# Autodesk Inventor assembly: Head
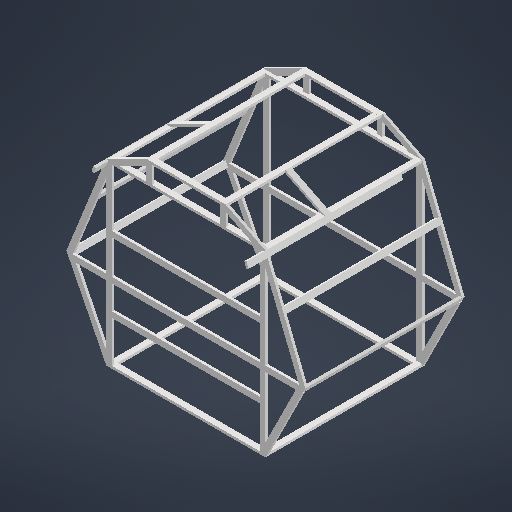
[picture p0: Inventor's stored thumbnail of the model, 512x512]
Saved by Autodesk Inventor 2026 (Build 300175000, 175)
## iProperties
Created: 2025-09-02
Part Number: Head
Document SubType Name: Assembly
Designer: trott
Author: trott
## Documents named in this file (12)
- C:\Users\trott\Documents\UofSC-ASME-Tiger-Burn-Design-2025\CAD\Head\Head.iam
- C:\Users\trott\Documents\UofSC-ASME-Tiger-Burn-Design-2025\CAD\Head\2x4x96.ipt
- C:\Users\trott\Documents\UofSC-ASME-Tiger-Burn-Design-2025\CAD\Head\2x4x89.ipt
- C:\Users\trott\Documents\UofSC-ASME-Tiger-Burn-Design-2025\CAD\Head\2x4x105.ipt
- C:\Users\trott\Documents\UofSC-ASME-Tiger-Burn-Design-2025\CAD\Head\S_2x4x24.ipt
- C:\Users\trott\Documents\UofSC-ASME-Tiger-Burn-Design-2025\CAD\Head\S_2x4x64.622.ipt
- C:\Users\trott\Documents\UofSC-ASME-Tiger-Burn-Design-2025\CAD\Head\S_2x4x48.13.ipt
- C:\Users\trott\Documents\UofSC-ASME-Tiger-Burn-Design-2025\CAD\Head\2x4x48.ipt
- C:\Users\trott\Documents\UofSC-ASME-Tiger-Burn-Design-2025\CAD\Head\2x4x10.5.ipt
- C:\Users\trott\Documents\UofSC-ASME-Tiger-Burn-Design-2025\CAD\Head\S_2x4x26.833.ipt
- C:\Users\trott\Documents\UofSC-ASME-Tiger-Burn-Design-2025\CAD\Head\2x4x93.ipt
- C:\Users\trott\Documents\UofSC-ASME-Tiger-Burn-Design-2025\CAD\Head\S2_2x4x26.833.ipt
## Components (48 placed, 11 different names)
1. 2x4x89:5 — Mate:5, Flush:11, Flush:12, Flush:14, Flush:15, Flush:18, Flush:23, Flush:24, Flush:49, Flush:52
2. 2x4x89:6 — Mate:6, Flush:13, Flush:14
3. S_2x4x64.622:1 — Mate:9, Flush:19
4. S_2x4x64.622:2 — Mate:10, Flush:20, Mate:46, Flush:58
5. S_2x4x64.622:3 — Mate:11, Mate:12, Flush:21, Mate:41, Mate:45, Flush:57
6. S_2x4x64.622:4 — Mate:13, Mate:14
7. S_2x4x48.13:1 — Mate:15, Flush:22, Mate:16
8. S_2x4x48.13:2 — Mate:17, Flush:25
9. S_2x4x48.13:3 — Mate:18, Mate:19, Flush:26, Mate:40
10. S_2x4x48.13:4 — Mate:20, Mate:21, Flush:27
11. 2x4x10.5:1 — Mate:22, Flush:28, Flush:32, Flush:39, Flush:40, Mate:27, Flush:46
12. 2x4x10.5:2 — Mate:23, Flush:29, Flush:31, Flush:45
13. 2x4x10.5:3 — Mate:24, Flush:34, Flush:35, Flush:38, Flush:47
14. 2x4x10.5:4 — Mate:25, Flush:33, Flush:36, Flush:37, Mate:26, Flush:48
15. 2x4x48:1 — Flush:37, Flush:38, Mate:26, Flush:41, Mate:28, Flush:42, Mate:33, Mate:35
16. 2x4x48:2 — Flush:39, Flush:40, Mate:27, Flush:43, Flush:44, Mate:29, Mate:30, Mate:31
17. 2x4x89:7 — Flush:41, Mate:28, Flush:42, Mate:43
18. 2x4x89:8 — Flush:43, Flush:44, Mate:29, Mate:42
19. S_2x4x26.833:1 — Flush:45, Mate:30, Flush:56
20. S_2x4x26.833:2 — Mate:31, Mate:32, Flush:46, Flush:55
21. S_2x4x26.833:3 — Mate:33, Mate:34, Flush:47
22. S_2x4x26.833:4 — Mate:35, Flush:48
23. 2x4x89:9 — Mate:36, Flush:49, Flush:50
24. 2x4x89:10 — Mate:37, Flush:51, Flush:52
25. 2x4x93:1 — Mate:38, Mate:39, Flush:53
26. 2x4x93:2 — Mate:40, Mate:41, Flush:54
27. S2_2x4x26.833:1 — Mate:42, Flush:56
28. S2_2x4x26.833:2 — Mate:43, Mate:44, Flush:55
29. 2x4x93:3 — Mate:45, Flush:57, Flush:64
30. 2x4x93:4 — Mate:46, Flush:58, Flush:63
31. 2x4x93:5 — Mate:51, Flush:63
32. 2x4x93:6 — Mate:52, Flush:64
33. 2x4x105:1 — Mate:4, Flush:9, Flush:10, Mate:5, Flush:11, Mate:8, Flush:17, Mate:19, Flush:26, Mate:36
34. 2x4x105:2 — Mate:6, Flush:13, Mate:20, Flush:27
35. 2x4x105:3 — Mate:7, Flush:16, Flush:22, Flush:50, Mate:37, Flush:51
36. 2x4x105:4 — Flush:25
37. 2x4x96:1 — Mate:1, Flush:1, Flush:2, Mate:2, Flush:3, Flush:4, Mate:4, Flush:9, Flush:10, Mate:21
38. 2x4x89:1 — Mate:1, Flush:1, Flush:2, Flush:8
39. 2x4x89:2 — Mate:2, Flush:3, Flush:4, Flush:5, Mate:3, Flush:6, Flush:7, Flush:12
40. 2x4x96:2 — Flush:5, Mate:3, Flush:6, Flush:7, Flush:8, Mate:15, Mate:16
41. 2x4x96:3 — Mate:12, Mate:13, Flush:32, Flush:35, Mate:32, Mate:34, Mate:44, Mate:52
42. 2x4x89:3 — Mate:24, Mate:25, Flush:33, Flush:34
43. 2x4x89:4 — Mate:22, Mate:23, Flush:28, Flush:29
44. 2x4x96:4 — Flush:31, Flush:36, Mate:51
45. S_2x4x24:2 — Mate:8, Flush:17, Flush:18, Mate:11, Flush:21, Flush:24, Mate:18, Flush:54
46. S_2x4x24:1 — Mate:7, Flush:15, Flush:16, Mate:10, Flush:20, Flush:23, Mate:38, Mate:39, Flush:53
47. S_2x4x24:3 — Mate:14
48. S_2x4x24:4 — Mate:9, Flush:19, Mate:17
## Component patterns: (4 elements, first: 2x4x105:1), (2 elements, first: 2x4x96:1 + 2x4x89:1 + 2x4x89:2 + 2x4x96:2), (2 elements, first: S_2x4x24:2 + S_2x4x24:1)
## Relationships (107: Flush 59, Mate 48)
- Mate:1: 2x4x96:1 ↔ 2x4x89:1
- Flush:1: 2x4x96:1 ↔ 2x4x89:1
- Flush:2: 2x4x96:1 ↔ 2x4x89:1
- Mate:2: 2x4x96:1 ↔ 2x4x89:2
- Flush:3: 2x4x96:1 ↔ 2x4x89:2
- Flush:4: 2x4x96:1 ↔ 2x4x89:2
- Flush:5: 2x4x89:2 ↔ 2x4x96:2
- Mate:3: 2x4x89:2 ↔ 2x4x96:2
- Flush:6: 2x4x89:2 ↔ 2x4x96:2
- Flush:7: 2x4x89:2 ↔ 2x4x96:2
- Flush:8: 2x4x89:1 ↔ 2x4x96:2
- Mate:4: 2x4x105:1 ↔ 2x4x96:1
- Flush:9: 2x4x105:1 ↔ 2x4x96:1
- Flush:10: 2x4x105:1 ↔ 2x4x96:1
- Mate:5: 2x4x89:5 ↔ 2x4x105:1
- Flush:11: 2x4x89:5 ↔ 2x4x105:1
- Flush:12 (1130.3 mm): 2x4x89:5 ↔ 2x4x89:2
- Mate:6: 2x4x89:6 ↔ 2x4x105:2
- Flush:13: 2x4x89:6 ↔ 2x4x105:2
- Flush:14: 2x4x89:5 ↔ 2x4x89:6
- Mate:7: 2x4x105:3 ↔ S_2x4x24:1
- Flush:15: 2x4x89:5 ↔ S_2x4x24:1
- Flush:16: 2x4x105:3 ↔ S_2x4x24:1
- Mate:8: 2x4x105:1 ↔ S_2x4x24:2
- Flush:17: 2x4x105:1 ↔ S_2x4x24:2
- Flush:18: 2x4x89:5 ↔ S_2x4x24:2
- Mate:9: S_2x4x64.622:1 ↔ S_2x4x24:4
- Flush:19: S_2x4x64.622:1 ↔ S_2x4x24:4
- Mate:10: S_2x4x64.622:2 ↔ S_2x4x24:1
- Flush:20: S_2x4x64.622:2 ↔ S_2x4x24:1
- Mate:11: S_2x4x64.622:3 ↔ S_2x4x24:2
- Mate:12: S_2x4x64.622:3 ↔ 2x4x96:3
- Flush:21: S_2x4x64.622:3 ↔ S_2x4x24:2
- Mate:13: S_2x4x64.622:4 ↔ 2x4x96:3
- Mate:14: S_2x4x64.622:4 ↔ S_2x4x24:3
- Mate:15: S_2x4x48.13:1 ↔ 2x4x96:2
- Flush:22: S_2x4x48.13:1 ↔ 2x4x105:3
- Mate:16: S_2x4x48.13:1 ↔ 2x4x96:2
- Flush:23: 2x4x89:5 ↔ S_2x4x24:1
- Flush:24: 2x4x89:5 ↔ S_2x4x24:2
- Mate:17: S_2x4x48.13:2 ↔ S_2x4x24:4
- Flush:25: S_2x4x48.13:2 ↔ 2x4x105:4
- Mate:18: S_2x4x48.13:3 ↔ S_2x4x24:2
- Mate:19: S_2x4x48.13:3 ↔ 2x4x105:1
- Flush:26: S_2x4x48.13:3 ↔ 2x4x105:1
- Mate:20: S_2x4x48.13:4 ↔ 2x4x105:2
- Mate:21: S_2x4x48.13:4 ↔ 2x4x96:1
- Flush:27: S_2x4x48.13:4 ↔ 2x4x105:2
- Mate:22: 2x4x10.5:1 ↔ 2x4x89:4
- Mate:23: 2x4x10.5:2 ↔ 2x4x89:4
- Flush:28: 2x4x10.5:1 ↔ 2x4x89:4
- Flush:29: 2x4x10.5:2 ↔ 2x4x89:4
- Flush:31 (609.6 mm): 2x4x10.5:2 ↔ 2x4x96:4
- Flush:32 (609.6 mm): 2x4x10.5:1 ↔ 2x4x96:3
- Mate:24: 2x4x10.5:3 ↔ 2x4x89:3
- Mate:25: 2x4x10.5:4 ↔ 2x4x89:3
- Flush:33: 2x4x10.5:4 ↔ 2x4x89:3
- Flush:34: 2x4x10.5:3 ↔ 2x4x89:3
- Flush:35 (609.6 mm): 2x4x10.5:3 ↔ 2x4x96:3
- Flush:36 (609.6 mm): 2x4x10.5:4 ↔ 2x4x96:4
- Flush:37: 2x4x10.5:4 ↔ 2x4x48:1
- Flush:38: 2x4x10.5:3 ↔ 2x4x48:1
- Mate:26: 2x4x10.5:4 ↔ 2x4x48:1
- Flush:39: 2x4x10.5:1 ↔ 2x4x48:2
- Flush:40: 2x4x10.5:1 ↔ 2x4x48:2
- Mate:27: 2x4x10.5:1 ↔ 2x4x48:2
- Flush:41: 2x4x48:1 ↔ 2x4x89:7
- Mate:28: 2x4x48:1 ↔ 2x4x89:7
- Flush:42: 2x4x48:1 ↔ 2x4x89:7
- Flush:43: 2x4x48:2 ↔ 2x4x89:8
- Flush:44: 2x4x48:2 ↔ 2x4x89:8
- Mate:29: 2x4x48:2 ↔ 2x4x89:8
- Flush:45: 2x4x10.5:2 ↔ S_2x4x26.833:1
- Mate:30: 2x4x48:2 ↔ S_2x4x26.833:1
- Mate:31: 2x4x48:2 ↔ S_2x4x26.833:2
- Mate:32: S_2x4x26.833:2 ↔ 2x4x96:3
- Flush:46: 2x4x10.5:1 ↔ S_2x4x26.833:2
- Mate:33: 2x4x48:1 ↔ S_2x4x26.833:3
- Mate:34: S_2x4x26.833:3 ↔ 2x4x96:3
- Flush:47: 2x4x10.5:3 ↔ S_2x4x26.833:3
- Mate:35: 2x4x48:1 ↔ S_2x4x26.833:4
- Flush:48: 2x4x10.5:4 ↔ S_2x4x26.833:4
- Mate:36: 2x4x89:9 ↔ 2x4x105:1
- Flush:49 (457.2 mm): 2x4x89:5 ↔ 2x4x89:9
- Flush:50: 2x4x89:9 ↔ 2x4x105:3
- Mate:37: 2x4x89:10 ↔ 2x4x105:3
- Flush:51: 2x4x89:10 ↔ 2x4x105:3
- Flush:52 (-609.6 mm): 2x4x89:5 ↔ 2x4x89:10
- Mate:38: 2x4x93:1 ↔ S_2x4x24:1
- Mate:39: 2x4x93:1 ↔ S_2x4x24:1
- Flush:53: 2x4x93:1 ↔ S_2x4x24:1
- Mate:40: S_2x4x48.13:3 ↔ 2x4x93:2
- Mate:41: S_2x4x64.622:3 ↔ 2x4x93:2
- Flush:54: 2x4x93:2 ↔ S_2x4x24:2
- Mate:42: 2x4x89:8 ↔ S2_2x4x26.833:1
- Mate:43: 2x4x89:7 ↔ S2_2x4x26.833:2
- Mate:44: S2_2x4x26.833:2 ↔ 2x4x96:3
- Flush:55 (914.4 mm): S_2x4x26.833:2 ↔ S2_2x4x26.833:2
- Flush:56 (914.4 mm): S_2x4x26.833:1 ↔ S2_2x4x26.833:1
- Mate:45: S_2x4x64.622:3 ↔ 2x4x93:3
- Flush:57: S_2x4x64.622:3 ↔ 2x4x93:3
- Mate:46: S_2x4x64.622:2 ↔ 2x4x93:4
- Flush:58: S_2x4x64.622:2 ↔ 2x4x93:4
- Mate:51: 2x4x93:5 ↔ 2x4x96:4
- Flush:63 (681.5582 mm): 2x4x93:4 ↔ 2x4x93:5
- Mate:52: 2x4x93:6 ↔ 2x4x96:3
- Flush:64 (681.5582 mm): 2x4x93:3 ↔ 2x4x93:6
